# Autodesk Inventor assembly: Kinematics
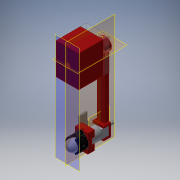
[picture p0: Inventor's stored thumbnail of the model, 180x180]
Saved by Autodesk Inventor 2019 (Build 230136000, 136)
## iProperties
Created: 2021-01-03
Part Number: Kinematics
Document SubType Name: Assembly
Designer: Sam
Author: Sam
## Documents named in this file (7)
- D:\OneDrive\MSc Robotics\GIC\RobotKinematics-Remote\3D CAD\Kinematics.iam
- D:\OneDrive\MSc Robotics\GIC\RobotKinematics-Remote\3D CAD\Base.ipt
- D:\OneDrive\MSc Robotics\GIC\RobotKinematics-Remote\3D CAD\Motor-GM15BY.iam
- D:\OneDrive\MSc Robotics\GIC\RobotKinematics-Remote\3D CAD\Base-Cover.ipt
- D:\OneDrive\MSc Robotics\GIC\RobotKinematics-Remote\3D CAD\Arm1.ipt
- D:\OneDrive\MSc Robotics\GIC\RobotKinematics-Remote\3D CAD\Mini-Q Ball caster.ipt
- D:\OneDrive\MSc Robotics\GIC\RobotKinematics-Remote\3D CAD\Arm1_BallCasterMount.ipt
## Components (7 placed, 6 different names)
1. Base:1 — Mate:1, Mate:2, Flush:1, Mate:14, Mate:15
2. Motor-GM15BY:1 [sub-assembly] — Mate:1, Mate:2, Mate:3, Mate:5, Mate:6
3. Base-Cover:1 — Flush:1, Mate:4, Mate:14, Mate:15
4. Arm1:1 — Mate:4, Mate:5, Mate:6, Mate:8, Mate:9, Mate:10
5. Motor-GM15BY:2 [sub-assembly] — Mate:8, Mate:9, Mate:10, Mate:11, Mate:12, Mate:13
6. Mini-Q Ball caster:1 — Tangent:1, Mate:11, Mate:12, Flush:2
7. Arm1_BallCasterMount:1 — Flush:2, Mate:13
## Relationships (17: Mate 14, Flush 2, Tangent 1)
- Mate:1: Base:1 ↔ Motor-GM15BY:1
- Mate:2: Base:1 ↔ Motor-GM15BY:1
- Mate:3: Motor-GM15BY:1
- Flush:1: Base:1 ↔ Base-Cover:1
- Mate:4 (2.5 mm): Base-Cover:1 ↔ Arm1:1
- Mate:5: Motor-GM15BY:1 ↔ Arm1:1
- Mate:6: Motor-GM15BY:1 ↔ Arm1:1
- Mate:8: Arm1:1 ↔ Motor-GM15BY:2
- Mate:9: Arm1:1 ↔ Motor-GM15BY:2
- Mate:10: Arm1:1 ↔ Motor-GM15BY:2
- Tangent:1: Mini-Q Ball caster:1
- Mate:11: Motor-GM15BY:2 ↔ Mini-Q Ball caster:1
- Mate:12: Motor-GM15BY:2 ↔ Mini-Q Ball caster:1
- Flush:2: Mini-Q Ball caster:1 ↔ Arm1_BallCasterMount:1
- Mate:13: Motor-GM15BY:2 ↔ Arm1_BallCasterMount:1
- Mate:14: Base:1 ↔ Base-Cover:1
- Mate:15: Base:1 ↔ Base-Cover:1
